# Autodesk Inventor assembly: Back Board Assembly
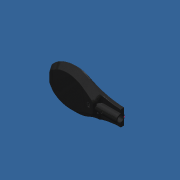
[picture p0: Inventor's stored thumbnail of the model, 180x180]
Saved by Autodesk Inventor 2018 (Build 220112000, 112)
## iProperties
Created: 2018-04-07
Part Number: Back Board Assembly
Document SubType Name: Assembly
Designer: Cole
Author: Cole
## Documents named in this file (3)
- D:\Cole\Documents\GitHub\SchoolCAD\ReverseEngineering\Back Board Assembly.iam
- D:\Cole\Documents\GitHub\SchoolCAD\ReverseEngineering\Back Board.ipt
- D:\Cole\Documents\GitHub\SchoolCAD\ReverseEngineering\Back Board Cover.ipt
## Components (2 placed, 2 different names)
1. Back Board:1 — Mate:1, Mate:2
2. Back Board Cover:1 — Mate:1, Mate:2
## Relationships (2: Mate 2)
- Mate:1: Back Board:1 ↔ Back Board Cover:1
- Mate:2: Back Board:1 ↔ Back Board Cover:1
